# Autodesk Inventor assembly: UpperArm
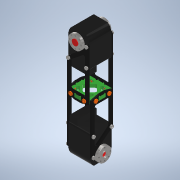
[picture p0: Inventor's stored thumbnail of the model, 180x180]
Saved by Autodesk Inventor 2020 (Build 240168000, 168)
## iProperties
Created: 2021-09-11
Part Number: UpperArm
Document SubType Name: Assembly
Designer: Masato
Mass: 132.402 g
Surface Area: 432.665 cm^2
Volume: 110.152 cm^3
Density: 1.20199 g/cm^3
Author: Masato
## Documents named in this file (12)
- C:\Users\MasatoKubotera\Documents\Inventor\OpenPlatform_ver3_0 - prototype\UpperBody\Arm\UpperArm.iam
- C:\Users\MasatoKubotera\Documents\Inventor\OpenPlatform_ver3_0 - prototype\UpperBody\Arm\UpperArm_side_frame.ipt
- C:\Users\MasatoKubotera\Documents\Inventor\OpenPlatform_ver3_0 - prototype\UpperBody\Arm\UpperArm_diagonal.ipt
- C:\Users\MasatoKubotera\Documents\Inventor\OpenPlatform_ver3_0 - prototype\ReadyMade\KONDO\B3M-SC-1040-A.ipt
- C:\Users\MasatoKubotera\Documents\Inventor\OpenPlatform_ver3_0 - prototype\ReadyMade\KONDO\FreeHorn.ipt
- C:\Users\MasatoKubotera\Documents\Inventor\OpenPlatform_ver3_0 - prototype\ReadyMade\Screw\M2_6-15.ipt
- C:\Users\MasatoKubotera\Documents\Inventor\OpenPlatform_ver3_0 - prototype\ReadyMade\Screw\M2_6-20.ipt
- C:\Users\MasatoKubotera\Documents\Inventor\OpenPlatform_ver3_0 - prototype\ReadyMade\Screw\M3-6.ipt
- C:\Users\MasatoKubotera\Documents\Inventor\OpenPlatform_ver3_0 - prototype\ReadyMade\KONDO\FreeHorn_Screw.ipt
- C:\Users\MasatoKubotera\Documents\Inventor\OpenPlatform_ver3_0 - prototype\ReadyMade\KONDO\ClampHorn.ipt
- C:\Users\MasatoKubotera\Documents\Inventor\OpenPlatform_ver3_0 - prototype\ReadyMade\InsertNut\IRU-304SW.ipt
- C:\Users\MasatoKubotera\Documents\Inventor\OpenPlatform_ver3_0 - prototype\ReadyMade\Screw\620103008.ipt
## Components (43 placed, 11 different names)
1. B3M-SC-1040-A:1 — 挿入:17, 挿入:18, 挿入:19, 挿入:20, 挿入:21, 挿入:22, 挿入:41, 挿入:45, 挿入:47, 角度:1, 挿入:73
2. ClampHorn:1 — 挿入:41, 角度:1, メイト:1
3. FreeHorn:2 — 挿入:46, メイト:2
4. B3M-SC-1040-A:2 — 挿入:42, 挿入:46, 挿入:48, 角度:2, 挿入:23, 挿入:24, 挿入:25, 挿入:26, 挿入:27, 挿入:28, 挿入:72
5. ClampHorn:2 — 挿入:42, 角度:2, メイト:2
6. FreeHorn:1 — 挿入:45, メイト:1
7. UpperArm_diagonal:1 — 挿入:1, 挿入:2, 挿入:3, 挿入:4, 挿入:5, 挿入:6, 挿入:7, 挿入:8, メイト:3, フラッシュ:1, フラッシュ:2, 挿入:64, 挿入:65, 挿入:66, 挿入:67, 挿入:68, 挿入:69, 挿入:70, 挿入:71
8. UpperArm_side_frame:1 — 挿入:1, 挿入:2, 挿入:9, 挿入:10, 挿入:23, 挿入:24, 挿入:25, 挿入:32, 挿入:33, 挿入:34
9. UpperArm_side_frame:2 — 挿入:3, 挿入:4, 挿入:11, 挿入:12, 挿入:26, 挿入:27, 挿入:28, 挿入:38, 挿入:39, 挿入:40
10. UpperArm_side_frame:3 — 挿入:8, 挿入:7, 挿入:14, 挿入:13, 挿入:17, 挿入:18, 挿入:19, 挿入:35, 挿入:36, 挿入:37
11. UpperArm_side_frame:4 — 挿入:6, 挿入:5, 挿入:15, 挿入:16, 挿入:20, 挿入:21, 挿入:22, 挿入:29, 挿入:30, 挿入:31
12. 620103008:1 — 挿入:73
13. 620103008:2 — 挿入:72
14. FreeHorn_Screw:1 — 挿入:47
15. FreeHorn_Screw:2 — 挿入:48
16. M2_6-20:6 — 挿入:40
17. M2_6-20:5 — 挿入:38
18. M2_6-20:4 — 挿入:39
19. M2_6-20:3 — 挿入:37
20. M2_6-20:2 — 挿入:36
21. M2_6-20:1 — 挿入:35
22. M2_6-15:6 — 挿入:34
23. M2_6-15:5 — 挿入:33
24. M2_6-15:4 — 挿入:32
25. M2_6-15:3 — 挿入:31
26. M2_6-15:2 — 挿入:30
27. M2_6-15:1 — 挿入:29
28. M3-6:8 — 挿入:16
29. M3-6:7 — 挿入:15
30. M3-6:6 — 挿入:14
31. M3-6:5 — 挿入:13
32. M3-6:4 — 挿入:12
33. M3-6:3 — 挿入:11
34. M3-6:2 — 挿入:10
35. M3-6:1 — 挿入:9
36. IRU-304SW:8 — 挿入:71
37. IRU-304SW:7 — 挿入:70
38. IRU-304SW:6 — 挿入:69
39. IRU-304SW:5 — 挿入:68
40. IRU-304SW:4 — 挿入:67
41. IRU-304SW:3 — 挿入:66
42. IRU-304SW:2 — 挿入:65
43. IRU-304SW:1 — 挿入:64
## Relationships (63: Insert 56, Mate 3, Angle 2, Flush 2)
- 挿入:1 [Insert]: UpperArm_diagonal:1 ↔ UpperArm_side_frame:1
- 挿入:2 [Insert]: UpperArm_diagonal:1 ↔ UpperArm_side_frame:1
- 挿入:3 [Insert]: UpperArm_diagonal:1 ↔ UpperArm_side_frame:2
- 挿入:4 [Insert]: UpperArm_diagonal:1 ↔ UpperArm_side_frame:2
- 挿入:5 [Insert]: UpperArm_diagonal:1 ↔ UpperArm_side_frame:4
- 挿入:6 [Insert]: UpperArm_diagonal:1 ↔ UpperArm_side_frame:4
- 挿入:7 [Insert]: UpperArm_diagonal:1 ↔ UpperArm_side_frame:3
- 挿入:8 [Insert]: UpperArm_diagonal:1 ↔ UpperArm_side_frame:3
- 挿入:11 [Insert]: UpperArm_side_frame:2 ↔ M3-6:3
- 挿入:12 [Insert]: UpperArm_side_frame:2 ↔ M3-6:4
- 挿入:13 [Insert]: UpperArm_side_frame:3 ↔ M3-6:5
- 挿入:14 [Insert]: UpperArm_side_frame:3 ↔ M3-6:6
- 挿入:15 [Insert]: UpperArm_side_frame:4 ↔ M3-6:7
- 挿入:16 [Insert]: UpperArm_side_frame:4 ↔ M3-6:8
- 挿入:17 [Insert]: B3M-SC-1040-A:1 ↔ UpperArm_side_frame:3
- 挿入:18 [Insert]: B3M-SC-1040-A:1 ↔ UpperArm_side_frame:3
- 挿入:19 [Insert]: B3M-SC-1040-A:1 ↔ UpperArm_side_frame:3
- 挿入:20 [Insert]: B3M-SC-1040-A:1 ↔ UpperArm_side_frame:4
- 挿入:21 [Insert]: B3M-SC-1040-A:1 ↔ UpperArm_side_frame:4
- 挿入:22 [Insert]: B3M-SC-1040-A:1 ↔ UpperArm_side_frame:4
- 挿入:29 [Insert]: UpperArm_side_frame:4 ↔ M2_6-15:1
- 挿入:30 [Insert]: UpperArm_side_frame:4 ↔ M2_6-15:2
- 挿入:31 [Insert]: UpperArm_side_frame:4 ↔ M2_6-15:3
- 挿入:32 [Insert]: UpperArm_side_frame:1 ↔ M2_6-15:4
- 挿入:33 [Insert]: UpperArm_side_frame:1 ↔ M2_6-15:5
- 挿入:35 [Insert]: UpperArm_side_frame:3 ↔ M2_6-20:1
- 挿入:34 [Insert]: UpperArm_side_frame:1 ↔ M2_6-15:6
- 挿入:36 [Insert]: UpperArm_side_frame:3 ↔ M2_6-20:2
- 挿入:37 [Insert]: UpperArm_side_frame:3 ↔ M2_6-20:3
- 挿入:9 [Insert]: UpperArm_side_frame:1 ↔ M3-6:1
- 挿入:10 [Insert]: UpperArm_side_frame:1 ↔ M3-6:2
- 挿入:38 [Insert]: UpperArm_side_frame:2 ↔ M2_6-20:5
- 挿入:39 [Insert]: UpperArm_side_frame:2 ↔ M2_6-20:4
- 挿入:40 [Insert]: UpperArm_side_frame:2 ↔ M2_6-20:6
- 挿入:41 [Insert]: B3M-SC-1040-A:1 ↔ ClampHorn:1
- 挿入:42 [Insert]: B3M-SC-1040-A:2 ↔ ClampHorn:2
- 挿入:45 [Insert]: B3M-SC-1040-A:1 ↔ FreeHorn:1
- 挿入:46 [Insert]: FreeHorn:2 ↔ B3M-SC-1040-A:2
- 挿入:47 [Insert]: B3M-SC-1040-A:1 ↔ FreeHorn_Screw:1
- 挿入:48 [Insert]: B3M-SC-1040-A:2 ↔ FreeHorn_Screw:2
- 角度:1 [Angle] (0 deg): B3M-SC-1040-A:1 ↔ ClampHorn:1
- 角度:2 [Angle] (0 deg): B3M-SC-1040-A:2 ↔ ClampHorn:2
- メイト:1 [Mate]: ClampHorn:1 ↔ FreeHorn:1
- メイト:2 [Mate]: FreeHorn:2 ↔ ClampHorn:2
- メイト:3 [Mate]: UpperArm_diagonal:1
- フラッシュ:1 [Flush]: UpperArm_diagonal:1
- フラッシュ:2 [Flush]: UpperArm_diagonal:1
- 挿入:23 [Insert]: B3M-SC-1040-A:2 ↔ UpperArm_side_frame:1
- 挿入:24 [Insert]: B3M-SC-1040-A:2 ↔ UpperArm_side_frame:1
- 挿入:25 [Insert]: B3M-SC-1040-A:2 ↔ UpperArm_side_frame:1
- 挿入:26 [Insert]: B3M-SC-1040-A:2 ↔ UpperArm_side_frame:2
- 挿入:27 [Insert]: B3M-SC-1040-A:2 ↔ UpperArm_side_frame:2
- 挿入:28 [Insert]: B3M-SC-1040-A:2 ↔ UpperArm_side_frame:2
- 挿入:64 [Insert]: UpperArm_diagonal:1 ↔ IRU-304SW:1
- 挿入:65 [Insert]: UpperArm_diagonal:1 ↔ IRU-304SW:2
- 挿入:66 [Insert]: UpperArm_diagonal:1 ↔ IRU-304SW:3
- 挿入:67 [Insert]: UpperArm_diagonal:1 ↔ IRU-304SW:4
- 挿入:68 [Insert]: UpperArm_diagonal:1 ↔ IRU-304SW:5
- 挿入:69 [Insert]: UpperArm_diagonal:1 ↔ IRU-304SW:6
- 挿入:70 [Insert]: UpperArm_diagonal:1 ↔ IRU-304SW:7
- 挿入:71 [Insert]: UpperArm_diagonal:1 ↔ IRU-304SW:8
- 挿入:72 [Insert]: B3M-SC-1040-A:2 ↔ 620103008:2
- 挿入:73 [Insert]: B3M-SC-1040-A:1 ↔ 620103008:1
